# Autodesk Inventor assembly: toit
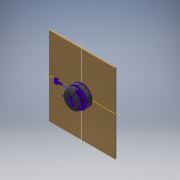
[picture p0: Inventor's stored thumbnail of the model, 180x180]
Saved by Autodesk Inventor 2019 (Build 230136000, 136)
## iProperties
Created: 2019-03-18
Part Number: toit
Document SubType Name: Assembly
Designer: franc
Author: franc
## Documents named in this file (3)
- C:\Users\franc\Desktop\EsialRobotik\Mecanique\2019\robot\toit.iam
- C:\Users\franc\Desktop\EsialRobotik\Mecanique\2019\robot\toit.ipt
- C:\Users\franc\Desktop\EsialRobotik\Mecanique\composants\RPlidar-A2M4\RPLIDAR A2.iam
## Components (2 placed, 2 different names)
1. toit:1 — Placage:1, Affleurement:1, Affleurement:2
2. RPLIDAR A2:1 [sub-assembly] — Placage:1, Placage:2, Placage:3, Placage:4
## Relationships (6: Mate 4, Flush 2)
- Placage:1 [Mate]: toit:1 ↔ RPLIDAR A2:1
- Affleurement:1 [Flush] (-150 mm): toit:1
- Affleurement:2 [Flush] (-125 mm): toit:1
- Placage:2 [Mate]: RPLIDAR A2:1
- Placage:3 [Mate]: RPLIDAR A2:1
- Placage:4 [Mate]: RPLIDAR A2:1
